# Autodesk Inventor assembly: IndexerPolyWheelPlateSet
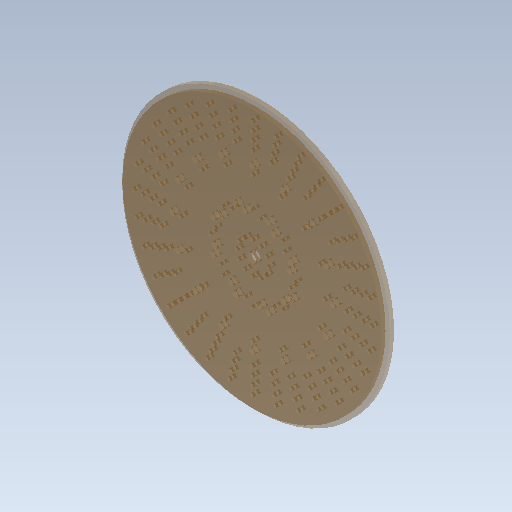
[picture p0: Inventor's stored thumbnail of the model, 512x512]
Saved by Autodesk Inventor 2020 (Build 240168000, 168)
## iProperties
Created: 2020-01-19
Part Number: IndexerPolyWheelPlateSet
Document SubType Name: Assembly
Designer: srini
Author: srini
## Documents named in this file (3)
- C:\Users\srini\Documents\FRC\2020\IntakeShooter\IndexerPolyWheelPlateSet.iam
- C:\Users\srini\Documents\FRC\2020\IntakeShooter\IndexWheelFlatPlatesPolyOutside.ipt
- C:\Users\srini\Documents\FRC\2020\IntakeShooter\IndexWheelFlatPlatesPolyInside.ipt
## Components (2 placed, 2 different names)
1. IndexWheelFlatPlatesPolyOutside:1 — Insert:1, Insert:2
2. IndexWheelFlatPlatesPolyInside:1 — Insert:1, Insert:2
## Relationships (2: Insert 2)
- Insert:1: IndexWheelFlatPlatesPolyOutside:1 ↔ IndexWheelFlatPlatesPolyInside:1
- Insert:2: IndexWheelFlatPlatesPolyOutside:1 ↔ IndexWheelFlatPlatesPolyInside:1
